# Autodesk Inventor assembly: outer
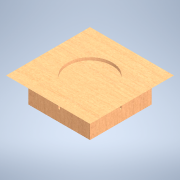
[picture p0: Inventor's stored thumbnail of the model, 180x180]
Saved by Autodesk Inventor 2021 (Build 250183000, 183)
## iProperties
Created: 2020-06-13
Part Number: outer
Document SubType Name: Assembly
Designer: Yatekii
Author: Yatekii
## Documents named in this file (5)
- C:\Users\Yatekii\repos\rcache\cad\outer.iam
- C:\Users\Yatekii\repos\rcache\cad\side.ipt
- C:\Users\Yatekii\repos\rcache\cad\inner_floor.ipt
- C:\Users\Yatekii\repos\rcache\cad\floor_side.ipt
- C:\Users\Yatekii\repos\rcache\cad\bottom.ipt
## Components (10 placed, 4 different names)
1. side:1 — Rigid:3
2. side:2 — Rigid:2, Rigid:3
3. side:3 — Rigid:1, Rigid:2
4. side:5 — Rigid:1, Rigid:6
5. inner_floor:1 — Mate:2, Flush:1, Mate:3, Mate:5
6. floor_side:1 — Mate:2, Flush:1, Mate:15, Mate:16, Mate:19
7. floor_side:2 — Flush:3, Mate:16, Mate:17, Flush:4, Mate:20
8. floor_side:3 — Mate:5, Mate:12, Flush:2, Flush:3, Mate:17, Flush:4, Mate:18
9. floor_side:4 — Mate:3, Mate:12, Mate:15, Flush:2
10. bottom:1 — Rigid:6, Mate:18, Mate:19, Mate:20
## Relationships (18: Mate 10, WeldJoint 4, Flush 4)
- Rigid:1 [WeldJoint]: side:3 ↔ side:5
- Rigid:2 [WeldJoint]: side:2 ↔ side:3
- Rigid:3 [WeldJoint]: side:1 ↔ side:2
- Mate:2: inner_floor:1 ↔ floor_side:1
- Flush:1: inner_floor:1 ↔ floor_side:1
- Mate:3: inner_floor:1 ↔ floor_side:4
- Mate:5: inner_floor:1 ↔ floor_side:3
- Rigid:6 [WeldJoint]: side:5 ↔ bottom:1
- Mate:12: floor_side:3 ↔ floor_side:4
- Mate:15: floor_side:1 ↔ floor_side:4
- Flush:2: floor_side:3 ↔ floor_side:4
- Flush:3: floor_side:2 ↔ floor_side:3
- Mate:16: floor_side:1 ↔ floor_side:2
- Mate:17: floor_side:2 ↔ floor_side:3
- Flush:4: floor_side:2 ↔ floor_side:3
- Mate:18: floor_side:3 ↔ bottom:1
- Mate:19 (10 mm): floor_side:1 ↔ bottom:1
- Mate:20 (10 mm): floor_side:2 ↔ bottom:1
